# Autodesk Inventor assembly: X-Carriage_LM3011
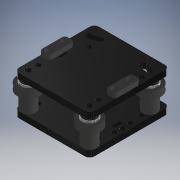
[picture p0: Inventor's stored thumbnail of the model, 180x180]
Saved by Autodesk Inventor 2020.2 (Build 242310000, 310)
## iProperties
Created: 2020-04-03
Part Number: X-Carriage_LM3011
Document SubType Name: Assembly
Designer: rah75
Author: rah75
## Documents named in this file (6)
- C:\Users\rah75\Documents\GitHub\LETU-Maker\CAD\Autodesk Inventor\Base_3001-5999\X-Carriage\Assemblies\X-Carriage_LM3011.iam
- C:\Users\rah75\Documents\GitHub\LETU-Maker\CAD\Autodesk Inventor\Base_3001-5999\X-Carriage\Fabricated_Parts\X-Carraige_Plate_LM3010.ipt
- C:\Users\rah75\Documents\GitHub\LETU-Maker\CAD\Autodesk Inventor\Base_3001-5999\X-Carriage\Printed_Parts\X-Carraige_Spacer_Long_LM3008.ipt
- C:\Users\rah75\Documents\GitHub\LETU-Maker\CAD\Autodesk Inventor\Base_3001-5999\X-Carriage\Printed_Parts\X-Carraige_Spacer_Short_LM3009.ipt
- C:\Users\rah75\Documents\GitHub\LETU-Maker\CAD\Autodesk Inventor\Base_3001-5999\X-Carriage\Printed_Parts\X-Carriage_Belt_Clamp_LM3007.ipt
- C:\Users\rah75\Documents\GitHub\LETU-Maker\CAD\Autodesk Inventor\Stock_Components_1001-2999\Power_Transmission\Bearings\V-Groove_Bearing_5mm_LM1041.ipt
## Components (16 placed, 5 different names)
1. X-Carraige_Plate_LM3010:1 — Insert:8, Insert:9, Insert:10, Insert:11, Insert:14, Insert:15, Mate:1, Mate:2
2. X-Carraige_Plate_LM3010:2 — Insert:13
3. X-Carraige_Spacer_Long_LM3008:1 — Insert:12
4. X-Carraige_Spacer_Short_LM3009:1 — Insert:4, Insert:9
5. X-Carraige_Spacer_Long_LM3008:2 — Insert:7
6. X-Carraige_Spacer_Short_LM3009:2 — Insert:3, Insert:8
7. X-Carraige_Spacer_Long_LM3008:3 — Insert:5, Insert:13
8. X-Carraige_Spacer_Short_LM3009:3 — Insert:2, Insert:11
9. X-Carraige_Spacer_Long_LM3008:4 — Insert:6
10. X-Carraige_Spacer_Short_LM3009:4 — Insert:1, Insert:10
11. X-Carriage_Belt_Clamp_LM3007:1 — Insert:15, Mate:2
12. X-Carriage_Belt_Clamp_LM3007:2 — Insert:14, Mate:1
13. V-Groove_Bearing_5mm_LM1041:1 — Insert:4, Insert:7
14. V-Groove_Bearing_5mm_LM1041:2 — Insert:3, Insert:5
15. V-Groove_Bearing_5mm_LM1041:3 — Insert:2, Insert:12
16. V-Groove_Bearing_5mm_LM1041:4 — Insert:1, Insert:6
## Relationships (17: Insert 15, Mate 2)
- Insert:1: X-Carraige_Spacer_Short_LM3009:4 ↔ V-Groove_Bearing_5mm_LM1041:4
- Insert:2: X-Carraige_Spacer_Short_LM3009:3 ↔ V-Groove_Bearing_5mm_LM1041:3
- Insert:3: X-Carraige_Spacer_Short_LM3009:2 ↔ V-Groove_Bearing_5mm_LM1041:2
- Insert:4: X-Carraige_Spacer_Short_LM3009:1 ↔ V-Groove_Bearing_5mm_LM1041:1
- Insert:5: X-Carraige_Spacer_Long_LM3008:3 ↔ V-Groove_Bearing_5mm_LM1041:2
- Insert:6: X-Carraige_Spacer_Long_LM3008:4 ↔ V-Groove_Bearing_5mm_LM1041:4
- Insert:7: X-Carraige_Spacer_Long_LM3008:2 ↔ V-Groove_Bearing_5mm_LM1041:1
- Insert:8: X-Carraige_Plate_LM3010:1 ↔ X-Carraige_Spacer_Short_LM3009:2
- Insert:9: X-Carraige_Plate_LM3010:1 ↔ X-Carraige_Spacer_Short_LM3009:1
- Insert:10: X-Carraige_Plate_LM3010:1 ↔ X-Carraige_Spacer_Short_LM3009:4
- Insert:11: X-Carraige_Plate_LM3010:1 ↔ X-Carraige_Spacer_Short_LM3009:3
- Insert:12: X-Carraige_Spacer_Long_LM3008:1 ↔ V-Groove_Bearing_5mm_LM1041:3
- Insert:13: X-Carraige_Plate_LM3010:2 ↔ X-Carraige_Spacer_Long_LM3008:3
- Insert:14: X-Carraige_Plate_LM3010:1 ↔ X-Carriage_Belt_Clamp_LM3007:2
- Insert:15: X-Carraige_Plate_LM3010:1 ↔ X-Carriage_Belt_Clamp_LM3007:1
- Mate:1: X-Carraige_Plate_LM3010:1 ↔ X-Carriage_Belt_Clamp_LM3007:2
- Mate:2: X-Carraige_Plate_LM3010:1 ↔ X-Carriage_Belt_Clamp_LM3007:1
